# Autodesk Inventor assembly: Assembly1
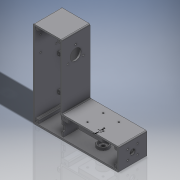
[picture p0: Inventor's stored thumbnail of the model, 180x180]
Saved by Autodesk Inventor 2019 (Build 230136000, 136)
## iProperties
Created: 2018-05-28
Part Number: Assembly1
Document SubType Name: Assembly
Designer: samps
Author: samps
## Documents named in this file (4)
- C:\Users\samps\Documents\Open Lidar\Open_Lidar_Hardware\Assembly1.iam
- C:\Users\samps\Documents\Open Lidar\Open_Lidar_Hardware\Main Lidar Body.ipt
- C:\Users\samps\Documents\Open Lidar\Open_Lidar_Hardware\Yaw Motor Mount.ipt
- C:\Users\samps\Documents\Open Lidar\Open_Lidar_Hardware\Yaw Shaft Mount.ipt
## Components (3 placed, 3 different names)
1. Main Lidar Body:1 — Mate:1, Flush:1, Mate:2, Mate:3
2. Yaw Motor Mount:1 — Mate:1, Flush:1
3. Yaw Shaft Mount:1 — Mate:2, Mate:4
## Relationships (6: Mate 5, Flush 1)
- Mate:1: Main Lidar Body:1 ↔ Yaw Motor Mount:1
- Flush:1: Main Lidar Body:1 ↔ Yaw Motor Mount:1
- Mate:2: Main Lidar Body:1 ↔ Yaw Shaft Mount:1
- Mate:3: Main Lidar Body:1
- Mate:4: Yaw Shaft Mount:1
- Mate:5
